# Autodesk Inventor assembly: XY gantry
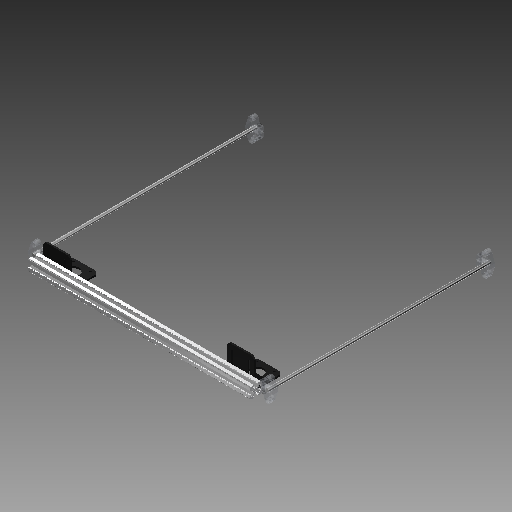
[picture p0: Inventor's stored thumbnail of the model, 512x512]
Saved by Autodesk Inventor 2017 SP1 (Build 210196100, 196)
## iProperties
Part Number: XY gantry
Material: Generisch
Document SubType Name: Assembly
Designer: Till
Author: Till
## Documents named in this file (5)
- C:\Users\Till\Dropbox\DIY\CoreBot\XY gantry.iam
- C:\Users\Till\Dropbox\DIY\CoreBot\CAD Parts\SHF8 x.ipt
- C:\Users\Till\Dropbox\DIY\CoreBot\CAD Parts\DriveLine 8x400mm.ipt
- C:\Users\Till\Dropbox\DIY\CoreBot\CAD Parts\Motor mount NEMA 17.ipt
- C:\Users\Till\Dropbox\DIY\CAD\400mm.ipt
## Components (9 placed, 4 different names)
1. SHF8 x:1 — Passend:4, Passend:9, Fluchtend:7, Fluchtend:9
2. SHF8 x:2 — Passend:5, Fluchtend:5, Fluchtend:7, Winkel:1
3. SHF8 x:3 — Passend:6, Passend:8, Fluchtend:6, Fluchtend:8
4. SHF8 x:4 — Passend:7, Fluchtend:4, Fluchtend:6, Winkel:2
5. DriveLine 8x400mm:1 — Passend:1, Fluchtend:3, Passend:6, Passend:7, Passend:8, Fluchtend:4, Passend:10, Passend:12
6. DriveLine 8x400mm:2 — Passend:1, Fluchtend:3, Passend:3, Passend:4, Passend:5, Passend:9, Fluchtend:5, Passend:11
7. Motor mount NEMA 17:1 — Passend:18
8. Motor mount NEMA 17:2 — Passend:19
9. 400mm:1 — Fluchtend:8, Fluchtend:9, Winkel:5, Passend:17, Fluchtend:10, Passend:18, Passend:19
## Relationships (25: Mate 14, Flush 8, Angle 3)
- Passend:1 [Mate] (420 mm): DriveLine 8x400mm:1 ↔ DriveLine 8x400mm:2
- Fluchtend:3 [Flush]: DriveLine 8x400mm:1 ↔ DriveLine 8x400mm:2
- Passend:3 [Mate]: DriveLine 8x400mm:2
- Passend:4 [Mate]: SHF8 x:1 ↔ DriveLine 8x400mm:2
- Passend:5 [Mate]: SHF8 x:2 ↔ DriveLine 8x400mm:2
- Passend:6 [Mate]: SHF8 x:3 ↔ DriveLine 8x400mm:1
- Passend:7 [Mate]: SHF8 x:4 ↔ DriveLine 8x400mm:1
- Passend:8 [Mate]: SHF8 x:3 ↔ DriveLine 8x400mm:1
- Passend:9 [Mate]: SHF8 x:1 ↔ DriveLine 8x400mm:2
- Fluchtend:4 [Flush]: SHF8 x:4 ↔ DriveLine 8x400mm:1
- Fluchtend:5 [Flush]: SHF8 x:2 ↔ DriveLine 8x400mm:2
- Passend:10 [Mate]: DriveLine 8x400mm:1
- Passend:11 [Mate]: DriveLine 8x400mm:2
- Passend:12 [Mate]: DriveLine 8x400mm:1
- Fluchtend:6 [Flush]: SHF8 x:3 ↔ SHF8 x:4
- Fluchtend:7 [Flush]: SHF8 x:1 ↔ SHF8 x:2
- Winkel:1 [Angle] (180 deg): SHF8 x:2
- Winkel:2 [Angle] (0 deg): SHF8 x:4
- Fluchtend:8 [Flush]: SHF8 x:3 ↔ 400mm:1
- Fluchtend:9 [Flush]: SHF8 x:1 ↔ 400mm:1
- Winkel:5 [Angle] (0 deg): 400mm:1
- Passend:17 [Mate]: 400mm:1
- Fluchtend:10 [Flush] (-10 mm): 400mm:1
- Passend:18 [Mate]: Motor mount NEMA 17:1 ↔ 400mm:1
- Passend:19 [Mate]: Motor mount NEMA 17:2 ↔ 400mm:1
